# Autodesk Inventor assembly: GearManipulator
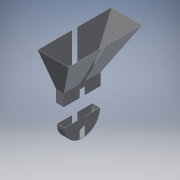
[picture p0: Inventor's stored thumbnail of the model, 180x180]
Saved by Autodesk Inventor 2016 (Build 200138000, 138)
## iProperties
Created: 2017-01-10
Part Number: GearManipulator
Document SubType Name: Assembly
Designer: hamblettk
Author: hamblettk
## Documents named in this file (3)
- F:\FRC\2017\2017Brainstorming\GearManipulator.iam
- F:\FRC\2017\2017Brainstorming\GearHolster.ipt
- F:\FRC\2017\2017Brainstorming\GearHopper.ipt
## Components (2 placed, 2 different names)
1. GearHolster:1 — Flush:1, Flush:2, Mate:1, Flush:3
2. GearHopper:1 — Flush:1, Flush:2, Mate:1, Flush:3
## Relationships (4: Flush 3, Mate 1)
- Flush:1: GearHolster:1 ↔ GearHopper:1
- Flush:2: GearHolster:1 ↔ GearHopper:1
- Mate:1 (152.4 mm): GearHolster:1 ↔ GearHopper:1
- Flush:3: GearHolster:1 ↔ GearHopper:1
